# Autodesk Inventor assembly: 5
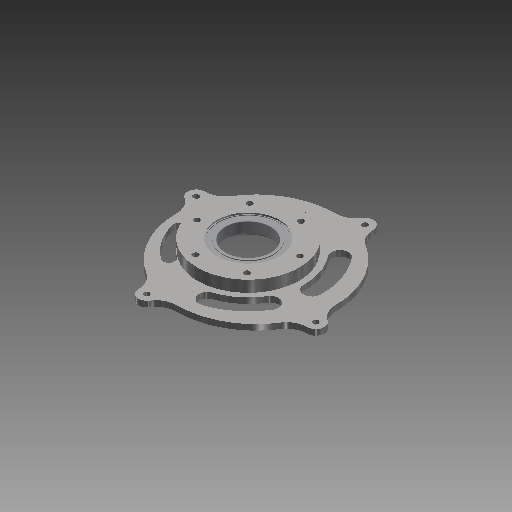
[picture p0: Inventor's stored thumbnail of the model, 512x512]
Saved by Autodesk Inventor 2019 (Build 230136000, 136)
## iProperties
Created: 2018-12-09
Part Number: 5
Document SubType Name: Assembly
Designer: steelen
Description: Small Eccentric Chain Tensioner
Material_size: As Specified
Quantity: 1
Author: steelen
## Documents named in this file (4)
- P:\me_fsae\2018_2019\ME\DriveTrain\Diff Parts\SmallEccentricChainTensioner.iam
- P:\me_fsae\2018_2019\ME\DriveTrain\Diff Parts\SmallBearingRing.ipt
- P:\me_fsae\2018_2019\ME\DriveTrain\Diff Parts\SKF61910-2RS1-Amazon.ipt
- P:\me_fsae\2018_2019\ME\DriveTrain\Diff Parts\SmallBearingPlate.ipt
## Components (3 placed, 3 different names)
1. SmallBearingRing:1 — Insert:1, Insert:2
2. SKF61910-2RS1-Amazon:1 — Insert:3
3. SmallBearingPlate:1 — Insert:1, Insert:2, Insert:3
## Relationships (3: Insert 3)
- Insert:1: SmallBearingRing:1 ↔ SmallBearingPlate:1
- Insert:2: SmallBearingRing:1 ↔ SmallBearingPlate:1
- Insert:3: SKF61910-2RS1-Amazon:1 ↔ SmallBearingPlate:1
